# Autodesk Inventor assembly: 275-1272
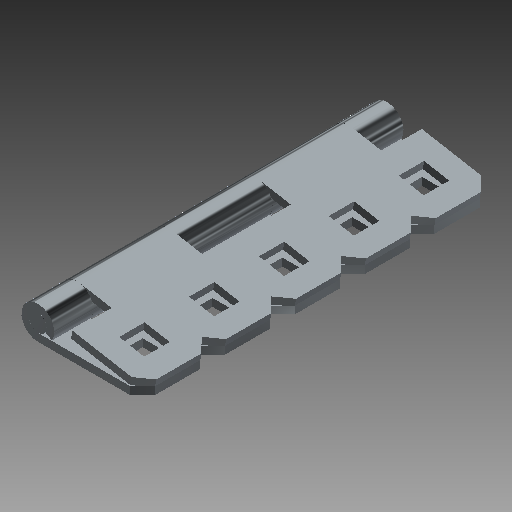
[picture p0: Inventor's stored thumbnail of the model, 512x512]
Saved by Autodesk Inventor 2018 (Build 220112000, 112)
## iProperties
Category: Structure
Company: Autodesk Inc.
Created: 2012-02-08
Part Number: 275-1272
Document SubType Name: Assembly
Designer: Autodesk Inc.
Catalog Web Link: http://www.vexrobotics.com/products/accessories/structure/275-1272.html
Vendor: VEX
Author: Autodesk Inc.
## Documents named in this file (4)
- C:\Users\USER\Desktop\School\Grade 12\Sem 1\Computer Engineering\Competition Robot Inventor\Vex Arm Assembly\Hinge.iam
- C:\Users\USER\Desktop\School\Grade 12\Sem 1\Computer Engineering\Competition Robot Inventor\Vex Arm Assembly\VEX-HINGE-1 RevA.ipt
- C:\Users\USER\Desktop\School\Grade 12\Sem 1\Computer Engineering\Competition Robot Inventor\Vex Arm Assembly\VEX-HINGE-2 RevA.ipt
- C:\Users\USER\Desktop\School\Grade 12\Sem 1\Computer Engineering\Competition Robot Inventor\Vex Arm Assembly\VEX-HINGE-PIN.ipt
## Components (3 placed, 3 different names)
1. VEX-HINGE-1 RevA:1 — Insert:1, Insert:2
2. VEX-HINGE-2 RevA:1 — Insert:1
3. VEX-HINGE-PIN:1 — Insert:2
## Relationships (2: Insert 2)
- Insert:1: VEX-HINGE-1 RevA:1 ↔ VEX-HINGE-2 RevA:1
- Insert:2: VEX-HINGE-1 RevA:1 ↔ VEX-HINGE-PIN:1
